# Autodesk Inventor assembly: mecanum wheel
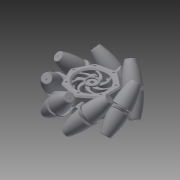
[picture p0: Inventor's stored thumbnail of the model, 180x180]
Saved by Autodesk Inventor 2015 (Build 190159000, 159)
## iProperties
Created: 2016-09-13
Part Number: mecanum wheel
Document SubType Name: Assembly
Designer: 294591
Title: 276-1447.STEP
Description: STEP AP203
Creation Date: 2011-11-15
Sending System: SolidWorks 2010
Preprocessor: SwSTEP 2.0
Author: 294591
## Documents named in this file (8)
- \\stushare\home\294591\Documents\Inventor\robotics\Imported Components\276-1447\mecanum wheel.iam
- \\stushare\home\294591\Documents\Inventor\robotics\Imported Components\276-1447\WHEEL.ipt
- \\stushare\home\294591\Documents\Inventor\robotics\Imported Components\276-1447\WASHER.ipt
- \\stushare\home\294591\Documents\Inventor\robotics\Imported Components\276-1447\SMALL-WHEEL-HUB.ipt
- \\stushare\home\294591\Documents\Inventor\robotics\Imported Components\276-1447\BRACKET-R.ipt
- \\stushare\home\294591\Documents\Inventor\robotics\Imported Components\276-1447\PIN.ipt
- \\stushare\home\294591\Documents\Inventor\robotics\Imported Components\276-1447\WHEEL-HUB-IN-R.ipt
- \\stushare\home\294591\Documents\Inventor\robotics\Imported Components\276-1447\WHEEL-HUB-OUT-R.ipt
## Components (58 placed, 58 different names)
1. WHEEL_1
2. WASHER_2
3. BRACKET-R_6
4. SMALL-WHEEL-HUB_7
5. PIN_8
6. WHEEL_9
7. WASHER_10
8. WHEEL_14
9. WASHER_15
10. BRACKET-R_19
11. PIN_20
12. WHEEL_21
13. WASHER_22
14. WHEEL_26
15. WASHER_27
16. BRACKET-R_32
17. BRACKET-R_33
18. SMALL-WHEEL-HUB_34
19. WHEEL_35
20. WASHER_36
21. WHEEL_40
22. WASHER_41
23. BRACKET-R_46
24. SMALL-WHEEL-HUB_47
25. WHEEL_48
26. WASHER_49
27. SMALL-WHEEL-HUB_53
28. SMALL-WHEEL-HUB_54
29. PIN_55
30. WASHER_56
31. BRACKET-R_61
32. SMALL-WHEEL-HUB_62
33. SMALL-WHEEL-HUB_63
34. WHEEL_64
35. WASHER_65
36. SMALL-WHEEL-HUB_69
37. PIN_70
38. WASHER_71
39. BRACKET-R_76
40. SMALL-WHEEL-HUB_77
41. WHEEL_78
42. WASHER_79
43. PIN_83
44. WHEEL-HUB-IN-R_84 — Flush:1
45. SMALL-WHEEL-HUB_89
46. SMALL-WHEEL-HUB_90
47. SMALL-WHEEL-HUB_91
48. WHEEL_92
49. WASHER_93
50. SMALL-WHEEL-HUB_97
51. PIN_98
52. WHEEL_99
53. SMALL-WHEEL-HUB_104
54. WHEEL_105
55. WASHER_106
56. WHEEL-HUB-OUT-R_110
57. PIN_111
58. WHEEL_112
## Relationships (1: Flush 1)
- Flush:1 (53.975 mm): WHEEL-HUB-IN-R_84
